# Autodesk Inventor assembly: Assembly1
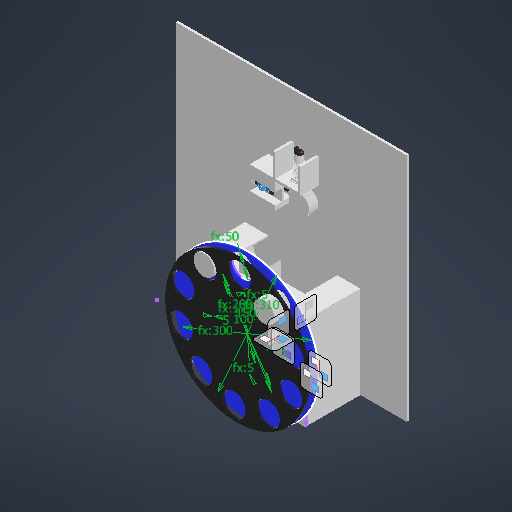
[picture p0: Inventor's stored thumbnail of the model, 512x512]
Saved by Autodesk Inventor 2027.1 (Build 311270010, 270A)
## iProperties
Created: 2026-09-28
Part Number: Assembly1
Document SubType Name: Assembly
Designer: daniel
Author: daniel
## Documents named in this file (11)
- C:\Users\danda\Desktop\Design 1\Project\CAD\Assembly1.iam
- C:\Users\danda\Desktop\Design 1\Project\CAD\Part2.ipt
- C:\Users\danda\Desktop\Design 1\Project\CAD\Part1.ipt
- C:\Users\danda\Desktop\Design 1\Project\CAD\base.ipt
- C:\Users\danda\Downloads\standard-servo-motor-black-1.snapshot.7\Assem1\Assem1.iam
- C:\Users\danda\Desktop\Design 1\Project\CAD\Part22.ipt
- C:\Users\danda\Desktop\Design 1\Project\CAD\Part23.ipt
- C:\Users\danda\Desktop\Design 1\Project\CAD\Part24.ipt
- C:\Users\danda\Desktop\Design 1\Project\CAD\Assembly7.iam
- C:\Users\danda\Desktop\Design 1\Project\CAD\Part27.ipt
- C:\Users\danda\Desktop\Design 1\Project\CAD\box\Assembly1.iam
## Components (10 placed, 10 different names)
1. Part2:1 — Mate:10, Tangent:1, Tangent:2, Mate:27
2. Part1:1 — Mate:8, Mate:9, Mate:10, Mate:15, Mate:16, Mate:31, Mate:32, Mate:34
3. base:1 — Mate:19, Flush:21, Mate:20, Mate:21, Flush:22, Flush:23
4. Assem1:1 [sub-assembly] — Mate:22, Mate:23, Mate:27, Mate:28, Mate:29, Mate:30, Mate:31
5. Part22:1 — Mate:8, Mate:9
6. Part23:1 — Tangent:1, Mate:15
7. Part24:1 — Mate:16, Tangent:2
8. Assembly7:1 [sub-assembly] — Mate:19, Flush:21
9. Part27:1 — Flush:24, Mate:33, Mate:34
10. Assembly1:1 [sub-assembly] — Mate:20, Mate:21, Flush:22, Flush:23, Mate:22, Mate:23, Mate:28, Mate:29, Mate:30, Mate:32, Flush:24, Mate:33
## Relationships (24: Mate 18, Flush 4, Tangent 2)
- Mate:8: Part1:1 ↔ Part22:1
- Mate:9: Part1:1 ↔ Part22:1
- Mate:10: Part2:1 ↔ Part1:1
- Tangent:1: Part2:1 ↔ Part23:1
- Mate:15: Part1:1 ↔ Part23:1
- Mate:16: Part1:1 ↔ Part24:1
- Tangent:2: Part2:1 ↔ Part24:1
- Mate:19: base:1 ↔ Assembly7:1
- Flush:21 (190 mm): base:1 ↔ Assembly7:1
- Mate:20: base:1 ↔ Assembly1:1
- Mate:21: base:1 ↔ Assembly1:1
- Flush:22: base:1 ↔ Assembly1:1
- Flush:23 (100 mm): base:1 ↔ Assembly1:1
- Mate:22: Assem1:1 ↔ Assembly1:1
- Mate:23: Assem1:1 ↔ Assembly1:1
- Mate:27: Part2:1 ↔ Assem1:1
- Mate:28: Assem1:1 ↔ Assembly1:1
- Mate:29: Assem1:1 ↔ Assembly1:1
- Mate:30: Assem1:1 ↔ Assembly1:1
- Mate:31: Part1:1 ↔ Assem1:1
- Mate:32: Part1:1 ↔ Assembly1:1
- Flush:24: Part27:1 ↔ Assembly1:1
- Mate:33: Part27:1 ↔ Assembly1:1
- Mate:34: Part1:1 ↔ Part27:1
